# Autodesk Inventor assembly: triangle_brace_mirrored
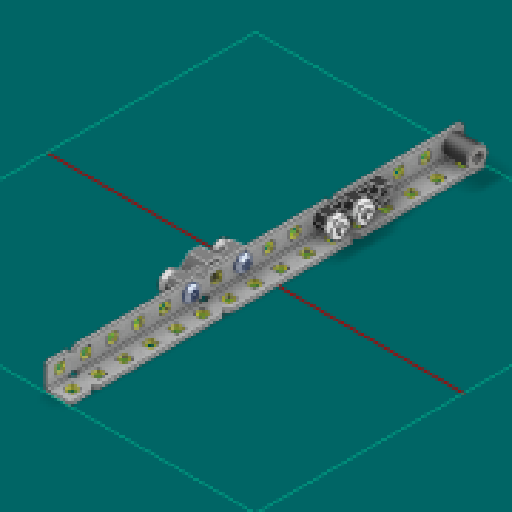
[picture p0: Inventor's stored thumbnail of the model, 512x512]
Saved by Autodesk Inventor 2025 (Build 290162000, 162)
## iProperties
Created: 2024-10-13
Part Number: triangle_brace_mirrored
Document SubType Name: Assembly
Designer: Averey Ku
Author: Averey Ku
## Documents named in this file (12)
- C:\Users\avere\vex_robotics_high_stakes\hardware\cad\bots\high_stakes_v2\tower\structure\side_mirrored\triangle_brace_mirrored.iam
- C:\Users\avere\vex_robotics_high_stakes\hardware\cad\bots\high_stakes_v2\tower\structure\side_mirrored\Alu Angle 1x1x16_mirrored.ipt
- C:\Users\avere\vex_robotics_high_stakes\hardware\cad\bots\high_stakes_v2\tower\structure\side_mirrored\HS Bearing Flat_mirrored.ipt
- C:\Users\avere\vex_robotics_high_stakes\hardware\cad\robpros_cad_lib\Motion\Spacers\Spacer Nylon .375 OD\NSpacer .375 OD x .500.ipt
- D:\vex_robotics_high_stakes\hardware\cad\robpros_cad_lib\Motion\Spacers\Spacer Nylon .375 OD.ipt
- C:\Users\avere\vex_robotics_high_stakes\hardware\cad\robpros_cad_lib\Motion\Spacers\Washer Steel\SWasher .375 OD x .015625.ipt
- D:\vex_robotics_high_stakes\hardware\cad\robpros_cad_lib\Motion\Spacers\Washer Steel.ipt
- C:\Users\avere\vex_robotics_high_stakes\hardware\cad\VEX-CAD-Inventor\Structure\Hardware\Screw Shoulder Robosource\SScrew Shoulder Smooth .500 x .04.ipt
- D:\vex_robotics_high_stakes\hardware\cad\VEX-CAD-Inventor\Structure\Hardware\Screw Shoulder Robosource.ipt
- C:\Users\avere\vex_robotics_high_stakes\hardware\cad\VEX-CAD-Inventor\Structure\Hardware\Nut Nylon\Nut Nylon - White.ipt
- D:\vex_robotics_high_stakes\hardware\cad\VEX-CAD-Inventor\Structure\Hardware\Nut Nylon.ipt
- C:\Users\avere\vex_robotics_high_stakes\hardware\cad\robpros_cad_lib\Quick Assemblies\bearing_flat_w_hardware_offset.iam
## Components (9 placed, 7 different names)
1. Alu Angle 1x1x16_mirrored:1 — Flush:1, Mate:3, Mate:2, Angle:1, Insert:1, Mate:1, Insert:4, Insert:5, Insert:7, Insert:9, Insert:10
2. HS Bearing Flat_mirrored:1 — Insert:1, Mate:1, Insert:11, Insert:12
3. NSpacer .375 OD x .500:1 — Insert:4, Insert:3
4. SWasher .375 OD x .015625:1 — Insert:3
5. SScrew Shoulder Smooth .500 x .04:1 — Insert:5, Mate:5
6. Nut Nylon - White:1 — Mate:5, Insert:11
7. SScrew Shoulder Smooth .500 x .04:2 — Insert:7, Mate:6
8. Nut Nylon - White:2 — Mate:6, Insert:12
9. bearing_flat_w_hardware_offset:1 [sub-assembly] — Insert:9, Insert:10
## Relationships (16: Insert 9, Mate 5, Flush 1, Angle 1)
- Flush:1: Alu Angle 1x1x16_mirrored:1
- Mate:3: Alu Angle 1x1x16_mirrored:1
- Mate:2 (6.35 mm): Alu Angle 1x1x16_mirrored:1
- Angle:1 (0 deg): Alu Angle 1x1x16_mirrored:1
- Insert:1: Alu Angle 1x1x16_mirrored:1 ↔ HS Bearing Flat_mirrored:1
- Mate:1: Alu Angle 1x1x16_mirrored:1 ↔ HS Bearing Flat_mirrored:1
- Insert:4: Alu Angle 1x1x16_mirrored:1 ↔ NSpacer .375 OD x .500:1
- Insert:3: NSpacer .375 OD x .500:1 ↔ SWasher .375 OD x .015625:1
- Insert:5: Alu Angle 1x1x16_mirrored:1 ↔ SScrew Shoulder Smooth .500 x .04:1
- Mate:5: SScrew Shoulder Smooth .500 x .04:1 ↔ Nut Nylon - White:1
- Insert:7: Alu Angle 1x1x16_mirrored:1 ↔ SScrew Shoulder Smooth .500 x .04:2
- Mate:6: SScrew Shoulder Smooth .500 x .04:2 ↔ Nut Nylon - White:2
- Insert:9: Alu Angle 1x1x16_mirrored:1 ↔ bearing_flat_w_hardware_offset:1
- Insert:10: Alu Angle 1x1x16_mirrored:1 ↔ bearing_flat_w_hardware_offset:1
- Insert:11: HS Bearing Flat_mirrored:1 ↔ Nut Nylon - White:1
- Insert:12: HS Bearing Flat_mirrored:1 ↔ Nut Nylon - White:2
